# Autodesk Inventor assembly: FullModHolder
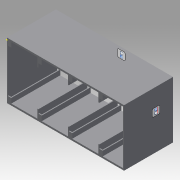
[picture p0: Inventor's stored thumbnail of the model, 180x180]
Saved by Autodesk Inventor 2016 (Build 200138000, 138)
## iProperties
Created: 2016-12-09
Part Number: FullModHolder
Document SubType Name: Assembly
Designer: Delta
Author: Delta
## Documents named in this file (3)
- C:\Robotics\CAD\2016-17_CAD\FullModHolder.iam
- C:\Robotics\CAD\2016-17_CAD\NewModuleHolder.ipt
- C:\Robotics\CAD\2016-17_CAD\NewModuleHolder Top.ipt
## Components (2 placed, 2 different names)
1. NewModuleHolder:1 — Flush:1, Flush:2, Mate:1
2. NewModuleHolder Top:1 — Flush:1, Flush:2, Mate:1
## Relationships (3: Flush 2, Mate 1)
- Flush:1: NewModuleHolder:1 ↔ NewModuleHolder Top:1
- Flush:2: NewModuleHolder:1 ↔ NewModuleHolder Top:1
- Mate:1 (89.408 mm): NewModuleHolder:1 ↔ NewModuleHolder Top:1
